# Autodesk Inventor assembly: Battery Box C Assembly
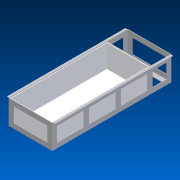
[picture p0: Inventor's stored thumbnail of the model, 180x180]
Saved by Autodesk Inventor 2012 (Build 160160000, 160)
## iProperties
Created: 2012-06-30
Part Number: Battery Box C Assembly
Document SubType Name: Assembly
Designer: Hemant
Author: Hemant
## Documents named in this file (10)
- C:\Users\Hemant\Documents\Battery Box C Assembly.iam
- C:\Users\Hemant\Documents\BOXC_L49.ipt
- C:\Users\Hemant\Documents\BOXC_L17P5.ipt
- C:\Users\Hemant\Documents\BOXC_F13P5.ipt
- C:\Users\Hemant\Documents\BOXC_F6.ipt
- C:\Users\Hemant\Documents\BOXC_L6.ipt
- C:\Users\Hemant\Documents\BOXC_F17P5.ipt
- C:\Users\Hemant\Documents\BOXC_L49_2.ipt
- C:\Users\Hemant\Documents\BOXC_F17P125.ipt
- C:\Users\Hemant\Documents\Plastic Box.iam
## Components (24 placed, 9 different names)
1. BOXC_L49:1 — Flush:1, Mate:1, Mate:2, Mate:3, Flush:4, Flush:8, Mate:7, Mate:8, Mate:9, Mate:15, Mate:16, Mate:17, Flush:11, Flush:12, Flush:13, Mate:18, Mate:24
2. BOXC_L49:2 — Flush:2, Flush:3, Mate:4, Mate:5, Mate:20, Mate:23, Flush:16, Mate:28, Flush:20, Mate:29, Flush:21, Mate:30, Flush:24
3. BOXC_L17P5:1 — Mate:2, Mate:3, Flush:4, Mate:5, Mate:19, Mate:21, Mate:25
4. BOXC_L17P5:2 — Flush:1, Mate:1, Flush:2, Flush:3, Mate:4, Flush:14, Mate:22, Flush:15
5. BOXC_F13P5:1 — Flush:5, Mate:9, Flush:16, Mate:25, Mate:26, Flush:17, Flush:22, Mate:40, Mate:44
6. BOXC_F13P5:2 — Flush:8, Mate:7, Mate:26, Mate:27, Flush:18, Flush:23
7. BOXC_F13P5:3 — Flush:5, Mate:8, Mate:27, Flush:19, Flush:25
8. BOXC_F6:1 — Mate:15, Flush:13, Flush:17
9. BOXC_F6:2 — Mate:16, Flush:12, Flush:18
10. BOXC_F6:3 — Mate:17, Flush:11, Flush:19
11. BOXC_L6:1 — Mate:20, Mate:21, Mate:31, Flush:27, Mate:35
12. BOXC_L6:2 — Mate:22, Flush:15, Mate:23, Mate:34
13. BOXC_L6:3 — Flush:14, Mate:24, Mate:33, Flush:28, Mate:37, Mate:38
14. BOXC_L6:4 — Mate:18, Mate:19, Mate:32
15. BOXC_F6:4 — Mate:28, Flush:20, Flush:22
16. BOXC_F6:5 — Mate:29, Flush:21, Flush:23
17. BOXC_F6:6 — Mate:30, Flush:24, Flush:25
18. BOXC_F17P5:1 — Mate:31, Flush:27, Mate:32, Mate:43
19. BOXC_F17P5:2 — Mate:33, Mate:34, Mate:36
20. BOXC_L49_2:1 — Flush:28, Mate:37, Mate:38, Flush:31
21. BOXC_L49_2:2 — Mate:35, Mate:36, Mate:42
22. BOXC_F17P125:1 — Flush:29, Mate:41, Flush:31, Mate:42, Mate:43
23. BOXC_F17P125:2 — Flush:29, Mate:40, Mate:41
24. Plastic Box:1 [sub-assembly] — Mate:44
## Relationships (62: Mate 37, Flush 25)
- Flush:1: BOXC_L49:1 ↔ BOXC_L17P5:2
- Mate:1: BOXC_L49:1 ↔ BOXC_L17P5:2
- Flush:2: BOXC_L49:2 ↔ BOXC_L17P5:2
- Flush:3: BOXC_L49:2 ↔ BOXC_L17P5:2
- Mate:2: BOXC_L49:1 ↔ BOXC_L17P5:1
- Mate:3: BOXC_L49:1 ↔ BOXC_L17P5:1
- Flush:4: BOXC_L49:1 ↔ BOXC_L17P5:1
- Mate:4: BOXC_L49:2 ↔ BOXC_L17P5:2
- Mate:5: BOXC_L49:2 ↔ BOXC_L17P5:1
- Flush:5: BOXC_F13P5:1 ↔ BOXC_F13P5:3
- Flush:8: BOXC_L49:1 ↔ BOXC_F13P5:2
- Mate:7: BOXC_L49:1 ↔ BOXC_F13P5:2
- Mate:8: BOXC_L49:1 ↔ BOXC_F13P5:3
- Mate:9: BOXC_L49:1 ↔ BOXC_F13P5:1
- Mate:15: BOXC_L49:1 ↔ BOXC_F6:1
- Mate:16: BOXC_L49:1 ↔ BOXC_F6:2
- Mate:17: BOXC_L49:1 ↔ BOXC_F6:3
- Flush:11: BOXC_L49:1 ↔ BOXC_F6:3
- Flush:12: BOXC_L49:1 ↔ BOXC_F6:2
- Flush:13: BOXC_L49:1 ↔ BOXC_F6:1
- Mate:18: BOXC_L49:1 ↔ BOXC_L6:4
- Mate:19: BOXC_L17P5:1 ↔ BOXC_L6:4
- Mate:20: BOXC_L49:2 ↔ BOXC_L6:1
- Mate:21: BOXC_L17P5:1 ↔ BOXC_L6:1
- Flush:14: BOXC_L17P5:2 ↔ BOXC_L6:3
- Mate:22: BOXC_L17P5:2 ↔ BOXC_L6:2
- Flush:15: BOXC_L17P5:2 ↔ BOXC_L6:2
- Mate:23: BOXC_L49:2 ↔ BOXC_L6:2
- Mate:24: BOXC_L49:1 ↔ BOXC_L6:3
- Flush:16: BOXC_L49:2 ↔ BOXC_F13P5:1
- Mate:25 (281.94 mm): BOXC_L17P5:1 ↔ BOXC_F13P5:1
- Mate:26 (281.94 mm): BOXC_F13P5:1 ↔ BOXC_F13P5:2
- Mate:27 (281.94 mm): BOXC_F13P5:2 ↔ BOXC_F13P5:3
- Flush:17: BOXC_F13P5:1 ↔ BOXC_F6:1
- Flush:18: BOXC_F13P5:2 ↔ BOXC_F6:2
- Flush:19: BOXC_F13P5:3 ↔ BOXC_F6:3
- Mate:28: BOXC_L49:2 ↔ BOXC_F6:4
- Flush:20: BOXC_L49:2 ↔ BOXC_F6:4
- Mate:29: BOXC_L49:2 ↔ BOXC_F6:5
- Flush:21: BOXC_L49:2 ↔ BOXC_F6:5
- Flush:22: BOXC_F13P5:1 ↔ BOXC_F6:4
- Flush:23: BOXC_F13P5:2 ↔ BOXC_F6:5
- Mate:30: BOXC_L49:2 ↔ BOXC_F6:6
- Flush:24: BOXC_L49:2 ↔ BOXC_F6:6
- Flush:25: BOXC_F13P5:3 ↔ BOXC_F6:6
- Mate:31: BOXC_L6:1 ↔ BOXC_F17P5:1
- Flush:27: BOXC_L6:1 ↔ BOXC_F17P5:1
- Mate:32: BOXC_L6:4 ↔ BOXC_F17P5:1
- Mate:33: BOXC_L6:3 ↔ BOXC_F17P5:2
- Mate:34: BOXC_L6:2 ↔ BOXC_F17P5:2
- Mate:35: BOXC_L6:1 ↔ BOXC_L49_2:2
- Mate:36: BOXC_F17P5:2 ↔ BOXC_L49_2:2
- Flush:28: BOXC_L6:3 ↔ BOXC_L49_2:1
- Mate:37: BOXC_L6:3 ↔ BOXC_L49_2:1
- Mate:38: BOXC_L6:3 ↔ BOXC_L49_2:1
- Flush:29: BOXC_F17P125:1 ↔ BOXC_F17P125:2
- Mate:40: BOXC_F13P5:1 ↔ BOXC_F17P125:2
- Mate:41: BOXC_F17P125:1 ↔ BOXC_F17P125:2
- Flush:31 (-6.7056 mm): BOXC_L49_2:1 ↔ BOXC_F17P125:1
- Mate:42: BOXC_L49_2:2 ↔ BOXC_F17P125:1
- Mate:43 (1022.35 mm): BOXC_F17P5:1 ↔ BOXC_F17P125:1
- Mate:44: BOXC_F13P5:1 ↔ Plastic Box:1
